# Autodesk Inventor assembly: Tape Measure Bracket Assembly V5
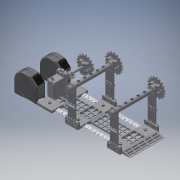
[picture p0: Inventor's stored thumbnail of the model, 180x180]
Saved by Autodesk Inventor 2019 (Build 230136000, 136)
## iProperties
Created: 2018-11-08
Part Number: Tape Measure Bracket Assembly V5
Document SubType Name: Assembly
Designer: Ashley
Author: Ashley
## Documents named in this file (35)
- C:\Users\Ashley\Desktop\repositories\design\inventor\2018-2019\Tape Measure Bracket\Version Six\Tape Measure Bracket Assembly V6.iam
- C:\Users\Ashley\Desktop\repositories\design\inventor\2018-2019\Tape Measure Bracket\Version Six\Bracket Bottom V6.ipt
- C:\Users\Ashley\Desktop\repositories\design\inventor\2018-2019\Tape Measure Bracket\Tape Measure\Tape Measure Edited.iam
- C:\Users\Ashley\Desktop\repositories\design\inventor\2018-2019\Tape Measure Bracket\Version Four\Side V4.ipt
- C:\Users\Ashley\Desktop\repositories\design\inventor\2018-2019\Tape Measure Bracket\Version Two\Braket Top V2.ipt
- C:\Users\Ashley\Desktop\repositories\design\inventor\2018-2019\Tape Measure Bracket\Version Five\Tape Measure Bracket Assembly V5\Design Accelerator\Bolted Connection2.iam
- C:\Users\Ashley\Desktop\repositories\design\inventor\2018-2019\Tape Measure Bracket\Version Five\Tape Measure Bracket Assembly V5\Design Accelerator\Bolted Connection3.iam
- C:\Users\Ashley\Desktop\repositories\design\inventor\2018-2019\Tape Measure Bracket\Version Five\Tape Measure Bracket Assembly V5\Design Accelerator\Bolted Connection4.iam
- C:\Users\Ashley\Desktop\repositories\design\inventor\2018-2019\Tape Measure Bracket\Version Five\Tape Measure Bracket Assembly V5\Design Accelerator\Bolted Connection6.iam
- C:\Users\Ashley\Desktop\repositories\design\inventor\2018-2019\Tape Measure Bracket\Version Five\Tape Measure Bracket Assembly V5\Design Accelerator\Bolted Connection7.iam
- C:\Users\Ashley\Desktop\repositories\design\inventor\2018-2019\Tape Measure Bracket\Version Five\Tape Measure Bracket Assembly V5\Design Accelerator\Bolted Connection8.iam
- C:\Users\Ashley\Desktop\repositories\design\inventor\2018-2019\Tape Measure Bracket\Version Five\Tape Measure Bracket Assembly V5\Design Accelerator\Bolted Connection9.iam
- C:\Users\Ashley\Desktop\repositories\design\inventor\2018-2019\Tape Measure Bracket\Version Five\Tape Measure Bracket Assembly V5\Design Accelerator\Bolted Connection10.iam
- C:\Users\Ashley\Desktop\repositories\design\inventor\2018-2019\Tape Measure Bracket\Version Five\Tape Measure Bracket Assembly V5\Design Accelerator\Bolted Connection11.iam
- C:\Users\Ashley\Desktop\repositories\design\inventor\2018-2019\Tape Measure Bracket\Version Five\Tape Measure Bracket Assembly V5\Design Accelerator\Bolted Connection12.iam
- C:\Users\Ashley\Desktop\repositories\design\inventor\2018-2019\Tape Measure Bracket\Version Five\Tape Measure Bracket Assembly V5\Design Accelerator\Bolted Connection13.iam
- C:\Users\Ashley\Desktop\repositories\design\inventor\Imported Components\goBilda\Bearing6mmID.ipt
- C:\Users\Ashley\Desktop\repositories\design\inventor\Imported Components\goBilda\Collar6mm\SetScrewCollar6mmboreassembly.iam
- C:\Users\Ashley\Desktop\repositories\design\inventor\Imported Components\goBilda\CampingHub\ClampingHub assembly.iam
- C:\Users\Ashley\Desktop\repositories\design\inventor\Imported Components\goBilda\8mmPlasticPitchSproket.ipt
- C:\Users\Ashley\Desktop\repositories\design\inventor\2018-2019\Tape Measure Bracket\Version Five\Tape Measure Bracket Assembly V5\Design Accelerator\Bolted Connection14.iam
- C:\Users\Ashley\Desktop\repositories\design\inventor\2018-2019\Tape Measure Bracket\Version Five\Tape Measure Bracket Assembly V5\Design Accelerator\Bolted Connection15.iam
- C:\Users\Ashley\Desktop\repositories\design\inventor\2018-2019\Tape Measure Bracket\Version Five\Tape Measure Bracket Assembly V5\Design Accelerator\Bolted Connection16.iam
- C:\Users\Ashley\Desktop\repositories\design\inventor\2018-2019\Tape Measure Bracket\Version Five\Tape Measure Bracket Assembly V5\Design Accelerator\Bolted Connection17.iam
- C:\Users\Ashley\Desktop\repositories\design\inventor\2018-2019\Tape Measure Bracket\Version Five\Tape Measure Bracket Assembly V5\Design Accelerator\Bolted Connection18.iam
- C:\Users\Ashley\Desktop\repositories\design\inventor\Imported Components\goBilda\Servo and Frame.iam
- C:\Users\Ashley\Desktop\repositories\design\inventor\Imported Components\goBilda\Servo To Shaft\ServoToShaftCoupler.iam
- C:\Users\Ashley\Desktop\repositories\design\inventor\2018-2019\Tape Measure Bracket\Version Five\Tape Measure Bracket Assembly V5\Design Accelerator\Bolted Connection20.iam
- C:\Users\Ashley\Desktop\repositories\design\inventor\Imported Components\goBilda\DShaft50mm.ipt
- C:\Users\Ashley\Desktop\repositories\design\inventor\2018-2019\Tape Measure Bracket\Version Six\Tape Measure Bracket Assembly V6\Design Accelerator\Bolted Connection1.iam
- C:\Users\Ashley\Desktop\repositories\design\inventor\2018-2019\Tape Measure Bracket\Version Six\Long Braket Top V6.ipt
- C:\Users\Ashley\Desktop\repositories\design\inventor\2018-2019\Tape Measure Bracket\Version Six\Tape Measure Bracket Assembly V6\Design Accelerator\Bolted Connection2.iam
- C:\Users\Ashley\Desktop\repositories\design\inventor\2018-2019\Tape Measure Bracket\Version Six\Tape Measure Bracket Assembly V6\Design Accelerator\Bolted Connection3.iam
- C:\Users\Ashley\Desktop\repositories\design\inventor\2018-2019\Tape Measure Bracket\Version Six\DShaft30mmV6.ipt
- C:\Users\Ashley\Desktop\repositories\design\inventor\2018-2019\Tape Measure Bracket\Version Six\SpinnerV6.ipt
## Components (58 placed, 16 different names)
1. Bracket Bottom — Mate:4, Mate:5, Insert:1, Insert:2, Insert:3, Insert:4, Insert:5, Insert:6, Insert:29, Insert:34, Mate:51, Insert:35, Insert:36
2. Tape Measure Right [sub-assembly]
3. Tape Measure Left [sub-assembly]
4. Braket Top V2:1 — Mate:5, Mate:22, Mate:23
5. Braket Top V2:2 — Mate:4, Mate:20, Mate:21
6. Braket Top V2:3 — Mate:26, Mate:27
7. Braket Top V2:4 — Mate:24, Mate:25
8. Side V4:1 — Insert:6, Mate:16, Mate:17, Mate:18, Mate:19, Insert:9
9. Side V4:2 — Insert:1, Insert:2, Mate:6, Mate:7, Insert:7
10. Side V4:3 — Insert:3, Insert:4, Mate:8, Mate:9, Mate:10, Mate:11, Mate:28
11. Side V4:4 — Insert:5, Mate:12, Mate:13, Mate:14, Mate:15, Insert:8
12. Bolted Connection:1 [sub-assembly] — Mate:6, Mate:7
13. Bolted Connection:2 [sub-assembly] — Mate:8, Mate:9
14. Bolted Connection:3 [sub-assembly] — Mate:10, Mate:11
15. Bolted Connection:4 [sub-assembly] — Mate:12, Mate:13
16. Bolted Connection:5 [sub-assembly] — Mate:14, Mate:15
17. Bolted Connection:6 [sub-assembly] — Mate:16, Mate:17
18. Bolted Connection:7 [sub-assembly] — Mate:18, Mate:19
19. Bolted Connection:8 [sub-assembly] — Mate:20, Mate:21
20. Bolted Connection:9 [sub-assembly] — Mate:22, Mate:23
21. Bolted Connection:10 [sub-assembly] — Mate:24, Mate:25
22. Bolted Connection:11 [sub-assembly] — Mate:26, Mate:27
23. Bearing6mmID:1 — Mate:28, Insert:37
24. Bearing6mmID:2 — Insert:8, Insert:40
25. Bearing6mmID:3 — Insert:7, Insert:24, Insert:39
26. Bearing6mmID:4 — Insert:9, Insert:42
27. SetScrewCollar6mmboreassembly:4 [sub-assembly] — Insert:38
28. SetScrewCollar6mmboreassembly:5 [sub-assembly] — Insert:41
29. ClampingHub assembly:3 [sub-assembly] — Insert:24, Insert:26
30. 8mmPlasticPitchSproket:1 — Insert:26, Mate:37, Mate:38
31. ClampingHub assembly:4 [sub-assembly] — Insert:43
32. 8mmPlasticPitchSproket:2 — Mate:29, Mate:30, Mate:31, Mate:32, Mate:33, Mate:34, Mate:35, Mate:36
33. Bolted Connection:12 [sub-assembly] — Mate:29, Mate:30
34. Bolted Connection:13 [sub-assembly] — Mate:31, Mate:32
35. Bolted Connection:14 [sub-assembly] — Mate:33, Mate:34
36. Bolted Connection:15 [sub-assembly] — Mate:35, Mate:36
37. Bolted Connection:16 [sub-assembly] — Mate:37, Mate:38
38. Servo and Frame:2 [sub-assembly] — Insert:29, Insert:30, Insert:34, Mate:52
39. ServoToShaftCoupler:1 [sub-assembly] — Insert:30, Mate:41, Mate:42, Insert:31
40. Bolted Connection:18 [sub-assembly] — Mate:41, Mate:42
41. DShaft50mm:1 — Insert:31, Insert:33
42. ClampingHub assembly:5 [sub-assembly] — Insert:33
43. 8mmPlasticPitchSproket:3
44. Bolted Connection:19 [sub-assembly]
45. Bolted Connection:20 [sub-assembly]
46. Bolted Connection:21 [sub-assembly]
47. Bolted Connection:22 [sub-assembly]
48. Bolted Connection:23 [sub-assembly] — Mate:51, Mate:52
49. Long Braket Top V6:1 — Insert:36, Mate:53, Mate:54
50. Long Braket Top V6:2 — Insert:35, Mate:55, Mate:56
51. Bolted Connection:24 [sub-assembly] — Mate:53, Mate:54
52. Bolted Connection:25 [sub-assembly] — Mate:55, Mate:56
53. DShaft30mmV6:1 — Insert:42, Insert:43, Insert:45
54. DShaft30mmV6:2 — Insert:39
55. DShaft30mmV6:3 — Insert:40, Insert:41
56. DShaft30mmV6:4 — Insert:37, Insert:38, Insert:44
57. SpinnerV6:1 — Insert:44
58. SpinnerV6:2 — Insert:45
## Relationships (80: Mate 51, Insert 29)
- Mate:4: Bracket Bottom ↔ Braket Top V2:2
- Mate:5: Bracket Bottom ↔ Braket Top V2:1
- Insert:1: Bracket Bottom ↔ Side V4:2
- Insert:2: Bracket Bottom ↔ Side V4:2
- Insert:3: Bracket Bottom ↔ Side V4:3
- Insert:4: Bracket Bottom ↔ Side V4:3
- Mate:6: Side V4:2 ↔ Bolted Connection:1
- Mate:7: Side V4:2 ↔ Bolted Connection:1
- Mate:8: Side V4:3 ↔ Bolted Connection:2
- Mate:9: Side V4:3 ↔ Bolted Connection:2
- Mate:10: Side V4:3 ↔ Bolted Connection:3
- Mate:11: Side V4:3 ↔ Bolted Connection:3
- Insert:5: Bracket Bottom ↔ Side V4:4
- Mate:12: Side V4:4 ↔ Bolted Connection:4
- Mate:13: Side V4:4 ↔ Bolted Connection:4
- Mate:14: Side V4:4 ↔ Bolted Connection:5
- Mate:15: Side V4:4 ↔ Bolted Connection:5
- Insert:6: Bracket Bottom ↔ Side V4:1
- Mate:16: Side V4:1 ↔ Bolted Connection:6
- Mate:17: Side V4:1 ↔ Bolted Connection:6
- Mate:18: Side V4:1 ↔ Bolted Connection:7
- Mate:19: Side V4:1 ↔ Bolted Connection:7
- Mate:20: Braket Top V2:2 ↔ Bolted Connection:8
- Mate:21: Braket Top V2:2 ↔ Bolted Connection:8
- Mate:22: Braket Top V2:1 ↔ Bolted Connection:9
- Mate:23: Braket Top V2:1 ↔ Bolted Connection:9
- Mate:24: Braket Top V2:4 ↔ Bolted Connection:10
- Mate:25: Braket Top V2:4 ↔ Bolted Connection:10
- Mate:26: Braket Top V2:3 ↔ Bolted Connection:11
- Mate:27: Braket Top V2:3 ↔ Bolted Connection:11
- Insert:7 (-3.55 mm): Side V4:2 ↔ Bearing6mmID:3
- Mate:28: Side V4:3 ↔ Bearing6mmID:1
- Insert:8 (-3.5 mm): Side V4:4 ↔ Bearing6mmID:2
- Insert:9 (-3.5 mm): Side V4:1 ↔ Bearing6mmID:4
- Insert:24 (0.5 mm): Bearing6mmID:3 ↔ ClampingHub assembly:3
- Insert:26 (-1 mm): ClampingHub assembly:3 ↔ 8mmPlasticPitchSproket:1
- [Insert] (-1 mm): ClampingHub assembly:4 ↔ 8mmPlasticPitchSproket:2
- Mate:29: 8mmPlasticPitchSproket:2 ↔ Bolted Connection:12
- Mate:30: 8mmPlasticPitchSproket:2 ↔ Bolted Connection:12
- Mate:31: 8mmPlasticPitchSproket:2 ↔ Bolted Connection:13
- Mate:32: 8mmPlasticPitchSproket:2 ↔ Bolted Connection:13
- Mate:33: 8mmPlasticPitchSproket:2 ↔ Bolted Connection:14
- Mate:34: 8mmPlasticPitchSproket:2 ↔ Bolted Connection:14
- Mate:35: 8mmPlasticPitchSproket:2 ↔ Bolted Connection:15
- Mate:36: 8mmPlasticPitchSproket:2 ↔ Bolted Connection:15
- Mate:37: 8mmPlasticPitchSproket:1 ↔ Bolted Connection:16
- Mate:38: 8mmPlasticPitchSproket:1 ↔ Bolted Connection:16
- Insert:29: Bracket Bottom ↔ Servo and Frame:2
- Insert:30: Servo and Frame:2 ↔ ServoToShaftCoupler:1
- Mate:41: ServoToShaftCoupler:1 ↔ Bolted Connection:18
- Mate:42: ServoToShaftCoupler:1 ↔ Bolted Connection:18
- Insert:31 (-10 mm): ServoToShaftCoupler:1 ↔ DShaft50mm:1
- [Insert] (-1 mm): ClampingHub assembly:5 ↔ 8mmPlasticPitchSproket:3
- [Mate]: 8mmPlasticPitchSproket:3 ↔ Bolted Connection:19
- [Mate]: 8mmPlasticPitchSproket:3 ↔ Bolted Connection:19
- [Mate]: 8mmPlasticPitchSproket:3 ↔ Bolted Connection:20
- [Mate]: 8mmPlasticPitchSproket:3 ↔ Bolted Connection:20
- [Mate]: 8mmPlasticPitchSproket:3 ↔ Bolted Connection:21
- [Mate]: 8mmPlasticPitchSproket:3 ↔ Bolted Connection:21
- [Mate]: 8mmPlasticPitchSproket:3 ↔ Bolted Connection:22
- [Mate]: 8mmPlasticPitchSproket:3 ↔ Bolted Connection:22
- Insert:33 (0.1 mm): DShaft50mm:1 ↔ ClampingHub assembly:5
- Insert:34: Bracket Bottom ↔ Servo and Frame:2
- Mate:51: Bracket Bottom ↔ Bolted Connection:23
- Mate:52: Servo and Frame:2 ↔ Bolted Connection:23
- Insert:35 (-6 mm): Bracket Bottom ↔ Long Braket Top V6:2
- Insert:36 (-6 mm): Bracket Bottom ↔ Long Braket Top V6:1
- Mate:53: Long Braket Top V6:1 ↔ Bolted Connection:24
- Mate:54: Long Braket Top V6:1 ↔ Bolted Connection:24
- Mate:55: Long Braket Top V6:2 ↔ Bolted Connection:25
- Mate:56: Long Braket Top V6:2 ↔ Bolted Connection:25
- Insert:37 (-13.5 mm): Bearing6mmID:1 ↔ DShaft30mmV6:4
- Insert:38 (-8 mm): SetScrewCollar6mmboreassembly:4 ↔ DShaft30mmV6:4
- Insert:39 (-13.5 mm): Bearing6mmID:3 ↔ DShaft30mmV6:2
- Insert:40 (-13.5 mm): Bearing6mmID:2 ↔ DShaft30mmV6:3
- Insert:41 (-8 mm): SetScrewCollar6mmboreassembly:5 ↔ DShaft30mmV6:3
- Insert:42 (-13.5 mm): Bearing6mmID:4 ↔ DShaft30mmV6:1
- Insert:43 (-9 mm): ClampingHub assembly:4 ↔ DShaft30mmV6:1
- Insert:44 (-15.5 mm): DShaft30mmV6:4 ↔ SpinnerV6:1
- Insert:45 (-11.6 mm): DShaft30mmV6:1 ↔ SpinnerV6:2
## Named parameters: d144_d143 = -1 mm, d163_d152 = 0 mm, d164_d153 = 0 mm, d165_d150 = 0 mm, d166_d151 = 0 mm, d167_d148 = 0 mm, d168_d149 = 0 mm, d169_d146 = 0 mm, d170_d147 = 0 mm, d172_d144_d143 = -1 mm
